# Autodesk Inventor assembly: SERVO CAJA
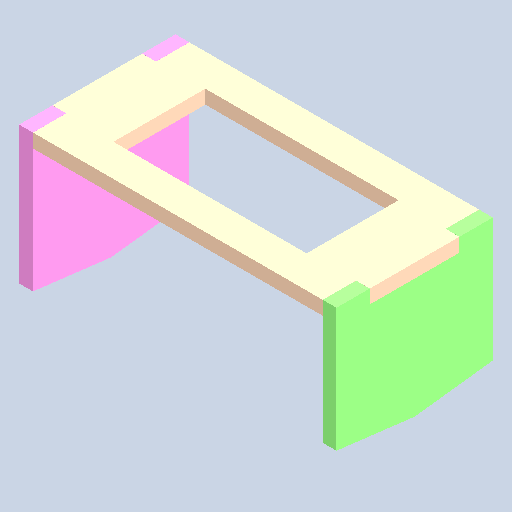
[picture p0: Inventor's stored thumbnail of the model, 512x512]
Saved by Autodesk Inventor 2025.3 (Build 293356030, 356C)
## iProperties
Created: 2025-07-09
Part Number: SERVO CAJA
Document SubType Name: Assembly
Designer: jv
Author: jv
## Documents named in this file (4)
- C:\Users\jv\Downloads\MODELOS NUEVOS\AILERON LINKAGE\SERVO CAJA.iam
- C:\Users\jv\Downloads\MODELOS NUEVOS\AILERON LINKAGE\B.ipt
- C:\Users\jv\Downloads\MODELOS NUEVOS\AILERON LINKAGE\A.ipt
- C:\Users\jv\Downloads\MODELOS NUEVOS\AILERON LINKAGE\C.ipt
## Components (3 placed, 3 different names)
1. B:1 — Mate:3, Mate:4
2. A:1 — Mate:1, Mate:2
3. C:1 — Mate:1, Mate:2, Mate:3, Mate:4
## Relationships (4: Mate 4)
- Mate:1: A:1 ↔ C:1
- Mate:2: A:1 ↔ C:1
- Mate:3: B:1 ↔ C:1
- Mate:4: B:1 ↔ C:1
